# Autodesk Inventor assembly: DriveTrain
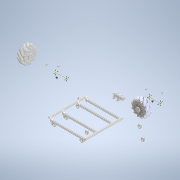
[picture p0: Inventor's stored thumbnail of the model, 180x180]
Saved by Autodesk Inventor 2020.2 (Build 242310000, 310)
## iProperties
Created: 2020-01-29
Part Number: DriveTrain
Document SubType Name: Assembly
Designer: yukin
Author: yukin
## Documents named in this file (16)
- C:\Autodesk\Files\CAD\Robotics 2019-2020\Assembly\DriveTrain\DriveTrain.iam
- C:\Autodesk\Files\CAD\Robotics 2019-2020\Assembly\DriveTrain\RevHexMotor\RevHexMotor.iam
- C:\Autodesk\Files\CAD\Robotics 2019-2020\Assembly\DriveTrain\MotorMount_vCAD.ipt
- C:\Autodesk\Files\CAD\Robotics 2019-2020\Assembly\DriveTrain\Extrusions\17in.ipt
- C:\Autodesk\Files\CAD\Robotics 2019-2020\Assembly\DriveTrain\CornerBracket.ipt
- C:\Autodesk\Files\CAD\Robotics 2019-2020\Assembly\DriveTrain\MotorMountBackSide.ipt
- C:\Autodesk\Files\CAD\Robotics 2019-2020\Assembly\DriveTrain\Extrusions\18in.ipt
- C:\Autodesk\Files\CAD\Robotics 2019-2020\Assembly\DriveTrain\BearingHolder.ipt
- C:\Autodesk\Files\CAD\Robotics 2019-2020\Assembly\DriveTrain\LMecaWheel\LMecaWheel.iam
- C:\Autodesk\Files\CAD\Robotics 2019-2020\Assembly\DriveTrain\RMecaWheel\RMecaWheel.iam
- C:\Autodesk\Files\CAD\Robotics 2019-2020\Assembly\DriveTrain\HexHub.ipt
- C:\Autodesk\Files\CAD\Robotics 2019-2020\Assembly\DriveTrain\WheelMount_v1_vCAD.ipt
- C:\Autodesk\Files\CAD\Robotics 2019-2020\Assembly\DriveTrain\WheelMount_v2_vCAD.ipt
- C:\Autodesk\Files\CAD\Robotics 2019-2020\Assembly\DriveTrain\HexShaft.ipt
- C:\Autodesk\Files\CAD\Robotics 2019-2020\Assembly\DriveTrain\ShaftCollar.ipt
- C:\Autodesk\Files\CAD\Robotics 2019-2020\Assembly\DriveTrain\Bearing.ipt
## Components (57 placed, 15 different names)
1. RevHexMotor:1 [sub-assembly] — Rotational:1, Insert:1
2. MotorMount_vCAD:1 — Rotational:1, Flush:21
3. 17in:1 — Flush:12, Flush:13, Mate:7, Mate:8, Flush:14, Flush:15, Mate:36, Flush:61, Flush:62, Mate:40, Flush:69, Flush:70
4. 17in:2 — Flush:8, Flush:9, Mate:5, Flush:10, Mate:6, Flush:11, Mate:34, Flush:57, Flush:58, Flush:67, Flush:68, Mate:39
5. CornerBracket:1 — Mate:35, Flush:59, Flush:60, Mate:36, Flush:61, Flush:62
6. CornerBracket:2 — Flush:55, Flush:56, Mate:33, Mate:34, Flush:57, Flush:58
7. CornerBracket:3 — Mate:8, Flush:14, Flush:15
8. CornerBracket:4 — Flush:12, Flush:13, Mate:7
9. CornerBracket:5 — Flush:8, Flush:9, Mate:5
10. CornerBracket:6 — Flush:10, Mate:6, Flush:11
11. CornerBracket:7 — Flush:67, Flush:68, Mate:39
12. CornerBracket:8 — Mate:40, Flush:69, Flush:70, Flush:71, Flush:72, Flush:73, Mate:41
13. MotorMountBackSide:1 — Insert:1, Flush:21
14. 18in:1 — Flush:71, Flush:72, Flush:73, Mate:41
15. 18in:2 — Flush:47, Flush:48, Mate:30, Mate:31, Flush:52, Flush:55, Flush:56, Mate:33, Mate:35, Flush:59, Flush:60
16. CornerBracket:9 — Mate:31, Flush:52, Mate:32, Flush:53, Flush:54
17. CornerBracket:10 — Flush:47, Flush:48, Mate:29, Flush:50, Flush:51, Mate:30
18. CornerBracket:11 — Flush:65, Mate:38, Flush:66
19. CornerBracket:12 — Flush:63, Mate:37, Flush:64
20. 17in:3 — Flush:39, Flush:40, Mate:24, Flush:43, Flush:44, Mate:26, Mate:29, Flush:49, Flush:50, Flush:51, Flush:63, Mate:37, Flush:64, Mate:45, Mate:48
21. 17in:4 — Mate:25, Flush:41, Flush:42, Flush:45, Flush:46, Mate:27, Mate:32, Flush:53, Flush:54, Flush:65, Mate:38, Flush:66, Mate:49, Flush:76
22. CornerBracket:13 — Flush:39, Flush:40, Mate:24, Flush:49, Mate:46, Flush:74
23. CornerBracket:14 — Flush:43, Flush:44, Mate:26, Mate:47, Flush:75
24. CornerBracket:15 — Mate:25, Flush:41, Flush:42
25. CornerBracket:16 — Flush:45, Flush:46, Mate:27, Mate:50
26. BearingHolder:1 — Mate:49, Mate:50, Flush:76
27. BearingHolder:2
28. BearingHolder:3
29. BearingHolder:4
30. LMecaWheel:2 [sub-assembly] — Insert:10, Insert:11, Insert:12, Insert:13
31. RMecaWheel:1 [sub-assembly] — Insert:2, Insert:3, Insert:6, Insert:7
32. HexHub:2 — Insert:8, Insert:9
33. HexHub:3 — Insert:4, Insert:5
34. WheelMount_v1_vCAD:1 — Insert:12, Insert:13
35. WheelMount_v1_vCAD:2 — Insert:6, Insert:7
36. WheelMount_v2_vCAD:1 — Insert:2, Insert:3, Insert:4, Insert:5
37. HexShaft:1
38. HexShaft:2 — Mate:43, Mate:44
39. WheelMount_v2_vCAD:2 — Insert:8, Insert:9, Insert:10, Insert:11
40. ShaftCollar:1 — Mate:44
41. ShaftCollar:2 — Mate:42
42. ShaftCollar:3
43. ShaftCollar:4
44. ShaftCollar:5
45. ShaftCollar:6
46. ShaftCollar:7
47. ShaftCollar:8
48. HexHub:4
49. HexHub:5
50. Bearing:1
51. Bearing:2
52. Bearing:3
53. Bearing:4
54. BearingHolder:5 — Mate:47, Mate:48, Flush:75
55. BearingHolder:6 — Mate:45, Mate:46, Flush:74
56. BearingHolder:7
57. BearingHolder:8
## Relationships (91: Flush 47, Mate 30, Insert 13, RevoluteJoint 1)
- Rotational:1 [RevoluteJoint]: RevHexMotor:1 ↔ MotorMount_vCAD:1
- Flush:8: 17in:2 ↔ CornerBracket:5
- Flush:9: 17in:2 ↔ CornerBracket:5
- Mate:5: 17in:2 ↔ CornerBracket:5
- Flush:10: 17in:2 ↔ CornerBracket:6
- Mate:6: 17in:2 ↔ CornerBracket:6
- Flush:11: 17in:2 ↔ CornerBracket:6
- Flush:12: 17in:1 ↔ CornerBracket:4
- Flush:13: 17in:1 ↔ CornerBracket:4
- Mate:7: 17in:1 ↔ CornerBracket:4
- Mate:8: 17in:1 ↔ CornerBracket:3
- Flush:14: 17in:1 ↔ CornerBracket:3
- Flush:15: 17in:1 ↔ CornerBracket:3
- Insert:1: RevHexMotor:1 ↔ MotorMountBackSide:1
- Flush:21: MotorMount_vCAD:1 ↔ MotorMountBackSide:1
- Flush:39: 17in:3 ↔ CornerBracket:13
- Flush:40: 17in:3 ↔ CornerBracket:13
- Mate:24: 17in:3 ↔ CornerBracket:13
- Mate:25: 17in:4 ↔ CornerBracket:15
- Flush:41: 17in:4 ↔ CornerBracket:15
- Flush:42: 17in:4 ↔ CornerBracket:15
- Flush:43: 17in:3 ↔ CornerBracket:14
- Flush:44: 17in:3 ↔ CornerBracket:14
- Mate:26: 17in:3 ↔ CornerBracket:14
- Flush:45: 17in:4 ↔ CornerBracket:16
- Flush:46: 17in:4 ↔ CornerBracket:16
- Mate:27: 17in:4 ↔ CornerBracket:16
- Insert:2: RMecaWheel:1 ↔ WheelMount_v2_vCAD:1
- Insert:3: RMecaWheel:1 ↔ WheelMount_v2_vCAD:1
- Insert:4: HexHub:3 ↔ WheelMount_v2_vCAD:1
- Insert:5: HexHub:3 ↔ WheelMount_v2_vCAD:1
- Insert:6: RMecaWheel:1 ↔ WheelMount_v1_vCAD:2
- Insert:7: RMecaWheel:1 ↔ WheelMount_v1_vCAD:2
- Insert:8: HexHub:2 ↔ WheelMount_v2_vCAD:2
- Insert:9: HexHub:2 ↔ WheelMount_v2_vCAD:2
- Insert:10: LMecaWheel:2 ↔ WheelMount_v2_vCAD:2
- Insert:11: LMecaWheel:2 ↔ WheelMount_v2_vCAD:2
- Insert:12: LMecaWheel:2 ↔ WheelMount_v1_vCAD:1
- Insert:13: LMecaWheel:2 ↔ WheelMount_v1_vCAD:1
- Flush:47: 18in:2 ↔ CornerBracket:10
- Flush:48: 18in:2 ↔ CornerBracket:10
- Mate:29: CornerBracket:10 ↔ 17in:3
- Flush:49: 17in:3 ↔ CornerBracket:13
- Flush:50: CornerBracket:10 ↔ 17in:3
- Flush:51: CornerBracket:10 ↔ 17in:3
- Mate:30: 18in:2 ↔ CornerBracket:10
- Mate:31: 18in:2 ↔ CornerBracket:9
- Flush:52: 18in:2 ↔ CornerBracket:9
- Mate:32: CornerBracket:9 ↔ 17in:4
- Flush:53: CornerBracket:9 ↔ 17in:4
- Flush:54: CornerBracket:9 ↔ 17in:4
- Flush:55: CornerBracket:2 ↔ 18in:2
- Flush:56: CornerBracket:2 ↔ 18in:2
- Mate:33: CornerBracket:2 ↔ 18in:2
- Mate:34: 17in:2 ↔ CornerBracket:2
- Flush:57: 17in:2 ↔ CornerBracket:2
- Flush:58: 17in:2 ↔ CornerBracket:2
- Mate:35: CornerBracket:1 ↔ 18in:2
- Flush:59: CornerBracket:1 ↔ 18in:2
- Flush:60: CornerBracket:1 ↔ 18in:2
- Mate:36: 17in:1 ↔ CornerBracket:1
- Flush:61: 17in:1 ↔ CornerBracket:1
- Flush:62: 17in:1 ↔ CornerBracket:1
- Flush:63: CornerBracket:12 ↔ 17in:3
- Mate:37: CornerBracket:12 ↔ 17in:3
- Flush:64: CornerBracket:12 ↔ 17in:3
- Flush:65: CornerBracket:11 ↔ 17in:4
- Mate:38: CornerBracket:11 ↔ 17in:4
- Flush:66: CornerBracket:11 ↔ 17in:4
- Flush:67: 17in:2 ↔ CornerBracket:7
- Flush:68: 17in:2 ↔ CornerBracket:7
- Mate:39: 17in:2 ↔ CornerBracket:7
- Mate:40: 17in:1 ↔ CornerBracket:8
- Flush:69: 17in:1 ↔ CornerBracket:8
- Flush:70: 17in:1 ↔ CornerBracket:8
- Flush:71: CornerBracket:8 ↔ 18in:1
- Flush:72: CornerBracket:8 ↔ 18in:1
- Flush:73: CornerBracket:8 ↔ 18in:1
- Mate:41: CornerBracket:8 ↔ 18in:1
- Mate:42: ShaftCollar:2
- Mate:43: HexShaft:2
- Mate:44: HexShaft:2 ↔ ShaftCollar:1
- Mate:45: 17in:3 ↔ BearingHolder:6
- Mate:46: CornerBracket:13 ↔ BearingHolder:6
- Flush:74: CornerBracket:13 ↔ BearingHolder:6
- Mate:47: CornerBracket:14 ↔ BearingHolder:5
- Mate:48: 17in:3 ↔ BearingHolder:5
- Flush:75: CornerBracket:14 ↔ BearingHolder:5
- Mate:49: 17in:4 ↔ BearingHolder:1
- Mate:50: CornerBracket:16 ↔ BearingHolder:1
- Flush:76: 17in:4 ↔ BearingHolder:1
